# Autodesk Inventor assembly: Battery Cage And Module
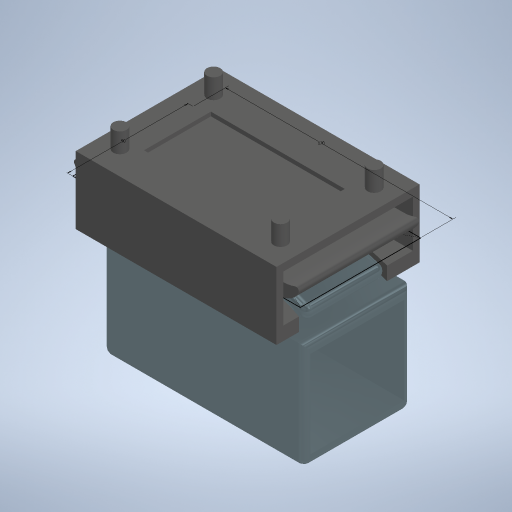
[picture p0: Inventor's stored thumbnail of the model, 512x512]
Saved by Autodesk Inventor 2023 (Build 270158000, 158)
## iProperties
Created: 2023-01-28
Part Number: Battery Cage And Module
Document SubType Name: Assembly
Designer: mihal
Author: mihal
## Documents named in this file (4)
- C:\Users\mihal\Desktop\Current BHSS Design\Eighth Assembly\Battery Cage And Module.iam
- C:\Users\mihal\Desktop\Current BHSS Design\Eighth Assembly\Battery Cage - Copy.ipt
- C:\Users\mihal\Desktop\Current BHSS Design\Eighth Assembly\Battery Container.ipt
- C:\Users\mihal\Desktop\Current BHSS Design\Eighth Assembly\Battery Cage Spring Plate.ipt
## Components (3 placed, 3 different names)
1. Battery Cage - Copy:1 — Mate:1, Mate:2, Mate:3, Mate:4, Mate:5
2. Battery Container:1 — Mate:1, Mate:2, Mate:3
3. Battery Cage Spring Plate:1 — Mate:4, Mate:5
## Relationships (5: Mate 5)
- Mate:1: Battery Cage - Copy:1 ↔ Battery Container:1
- Mate:2: Battery Cage - Copy:1 ↔ Battery Container:1
- Mate:3: Battery Cage - Copy:1 ↔ Battery Container:1
- Mate:4: Battery Cage - Copy:1 ↔ Battery Cage Spring Plate:1
- Mate:5: Battery Cage - Copy:1 ↔ Battery Cage Spring Plate:1
